# Autodesk Inventor assembly: Inner rails
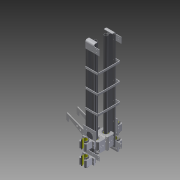
[picture p0: Inventor's stored thumbnail of the model, 180x180]
Saved by Autodesk Inventor 2013 (Build 170138000, 138)
## iProperties
Created: 2013-01-27
Part Number: Inner rails
Document SubType Name: Assembly
Designer: Arpan
Mass: 4602.07 g
Surface Area: 8094.53 cm^2
Volume: 1948.66 cm^3
Density: 2.36166 g/cm^3
Author: Arpan
## Documents named in this file (9)
- C:\Users\Arpan\Documents\GitHub\frc2013CAD\Cimber actual\Inner rails.iam
- C:\Users\Arpan\Documents\GitHub\frc2013CAD\Cimber actual\Shaft 26 inch.ipt
- C:\Users\Arpan\Documents\GitHub\frc2013CAD\Cimber actual\endstop.ipt
- C:\Users\Arpan\Documents\GitHub\frc2013CAD\Cimber actual\endstop 2.ipt
- C:\Users\Arpan\Documents\GitHub\frc2013CAD\Cimber actual\tie-together tier 1.ipt
- C:\Users\Arpan\Documents\GitHub\frc2013CAD\Cimber actual\upper face mount.ipt
- C:\Users\Arpan\Documents\GitHub\frc2013CAD\Cimber actual\face mount.ipt
- C:\Users\Arpan\Documents\GitHub\frc2013CAD\Cimber actual\bearing block short style.iam
- C:\Users\Arpan\Documents\GitHub\frc2013CAD\Cimber actual\hook block.iam
## Components (16 placed, 8 different names)
1. Shaft 26 inch:1 — Angle:1, Flush:1, Mate:2, Mate:6, Mate:7, Mate:8, Mate:9, Mate:10, Mate:15, Mate:16, Mate:17, Mate:18, Mate:19, Mate:22, Mate:23, Mate:31, Mate:32, Mate:47
2. Shaft 26 inch:2 — Angle:1, Flush:1, Mate:3, Mate:4, Mate:5, Mate:12, Mate:13, Mate:25, Mate:26, Mate:28, Mate:29, Mate:46, Flush:2
3. endstop:1 — Mate:2, Mate:6, Mate:7
4. endstop 2:1 — Mate:3, Mate:4, Mate:5
5. tie-together tier 1:1 — Mate:8, Mate:9, Mate:10, Mate:12, Mate:13
6. tie-together tier 1:2 — Mate:15, Mate:16, Mate:17
7. tie-together tier 1:3 — Mate:18, Mate:19
8. upper face mount:1 — Mate:25, Mate:26, Mate:42, Mate:43, Mate:44
9. upper face mount:2 — Mate:22, Mate:23, Mate:39, Mate:40, Mate:41
10. face mount:1 — Mate:28, Mate:29, Mate:36, Mate:37, Mate:38
11. face mount:2 — Mate:31, Mate:32, Mate:33, Mate:34, Mate:35
12. bearing block short style:1 [sub-assembly] — Mate:33, Mate:34, Mate:35
13. bearing block short style:2 [sub-assembly] — Mate:36, Mate:37, Mate:38
14. bearing block short style:3 [sub-assembly] — Mate:39, Mate:40, Mate:41
15. bearing block short style:4 [sub-assembly] — Mate:42, Mate:43, Mate:44
16. hook block:1 [sub-assembly] — Mate:46, Mate:47, Flush:2
## Relationships (41: Mate 38, Flush 2, Angle 1)
- Angle:1 (180 deg): Shaft 26 inch:1 ↔ Shaft 26 inch:2
- Flush:1: Shaft 26 inch:1 ↔ Shaft 26 inch:2
- Mate:2: Shaft 26 inch:1 ↔ endstop:1
- Mate:3: Shaft 26 inch:2 ↔ endstop 2:1
- Mate:4: Shaft 26 inch:2 ↔ endstop 2:1
- Mate:5: Shaft 26 inch:2 ↔ endstop 2:1
- Mate:6: Shaft 26 inch:1 ↔ endstop:1
- Mate:7: Shaft 26 inch:1 ↔ endstop:1
- Mate:8: Shaft 26 inch:1 ↔ tie-together tier 1:1
- Mate:9: Shaft 26 inch:1 ↔ tie-together tier 1:1
- Mate:10: Shaft 26 inch:1 ↔ tie-together tier 1:1
- Mate:12: Shaft 26 inch:2 ↔ tie-together tier 1:1
- Mate:13: Shaft 26 inch:2 ↔ tie-together tier 1:1
- Mate:15: Shaft 26 inch:1 ↔ tie-together tier 1:2
- Mate:16: Shaft 26 inch:1 ↔ tie-together tier 1:2
- Mate:17: Shaft 26 inch:1 ↔ tie-together tier 1:2
- Mate:18: Shaft 26 inch:1 ↔ tie-together tier 1:3
- Mate:19: Shaft 26 inch:1 ↔ tie-together tier 1:3
- Mate:22: Shaft 26 inch:1 ↔ upper face mount:2
- Mate:23: Shaft 26 inch:1 ↔ upper face mount:2
- Mate:25: Shaft 26 inch:2 ↔ upper face mount:1
- Mate:26: Shaft 26 inch:2 ↔ upper face mount:1
- Mate:28: Shaft 26 inch:2 ↔ face mount:1
- Mate:29: Shaft 26 inch:2 ↔ face mount:1
- Mate:31: Shaft 26 inch:1 ↔ face mount:2
- Mate:32: Shaft 26 inch:1 ↔ face mount:2
- Mate:33: face mount:2 ↔ bearing block short style:1
- Mate:34: face mount:2 ↔ bearing block short style:1
- Mate:35: face mount:2 ↔ bearing block short style:1
- Mate:36: face mount:1 ↔ bearing block short style:2
- Mate:37: face mount:1 ↔ bearing block short style:2
- Mate:38: face mount:1 ↔ bearing block short style:2
- Mate:39: upper face mount:2 ↔ bearing block short style:3
- Mate:40: upper face mount:2 ↔ bearing block short style:3
- Mate:41: upper face mount:2 ↔ bearing block short style:3
- Mate:42: upper face mount:1 ↔ bearing block short style:4
- Mate:43: upper face mount:1 ↔ bearing block short style:4
- Mate:44: upper face mount:1 ↔ bearing block short style:4
- Mate:46: Shaft 26 inch:2 ↔ hook block:1
- Mate:47: Shaft 26 inch:1 ↔ hook block:1
- Flush:2 (12.7 mm): Shaft 26 inch:2 ↔ hook block:1
